# Autodesk Inventor assembly: 2200_Coil Housing
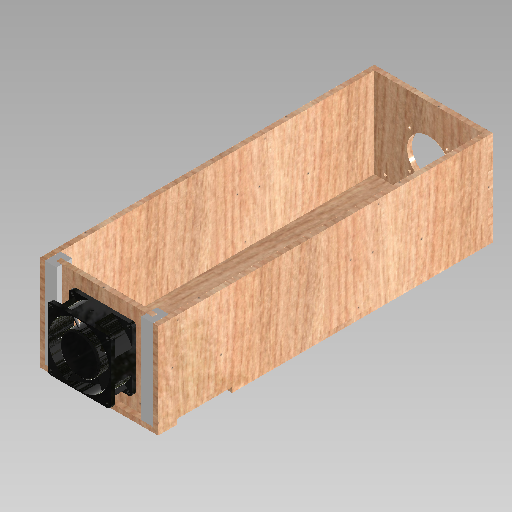
[picture p0: Inventor's stored thumbnail of the model, 512x512]
Saved by Autodesk Inventor 2020 (Build 240168000, 168)
## iProperties
Created: 2019-11-08
Part Number: 2200_Coil Housing
Document SubType Name: Assembly
Designer: RFLab
Author: RFLab
## Documents named in this file (7)
- C:\Users\e22ma\Dropbox\MPI Group Folder\MPS\Inventor_Parts\Parts Numbered - OSMPI\2xxx_Sample Holder and Rx\22xx_Coil Housing\2200_Coil Housing.iam
- C:\Users\e22ma\Dropbox\MPI Group Folder\MPS\Inventor_Parts\Parts Numbered - OSMPI\2xxx_Sample Holder and Rx\22xx_Coil Housing\2204_Housing Front_V1.ipt
- C:\Users\e22ma\Dropbox\MPI Group Folder\MPS\Inventor_Parts\Parts Numbered - OSMPI\2xxx_Sample Holder and Rx\22xx_Coil Housing\2202_Housing Side_V1.ipt
- C:\Users\e22ma\Dropbox\MPI Group Folder\MPS\Inventor_Parts\Parts Numbered - OSMPI\2xxx_Sample Holder and Rx\22xx_Coil Housing\2203_Housing Back.ipt
- C:\Users\e22ma\Dropbox\MPI Group Folder\MPS\Inventor_Parts\Parts Numbered - OSMPI\2xxx_Sample Holder and Rx\22xx_Coil Housing\2208_Back Plate Groove_V1.ipt
- C:\Users\e22ma\Dropbox\MPI Group Folder\MPS\Inventor_Parts\Parts Numbered - OSMPI\2xxx_Sample Holder and Rx\22xx_Coil Housing\2201_Housing Bottom_V1.ipt
- C:\Users\e22ma\Dropbox\MPI Student Access\Helpful Files\Inventor\DC EQUIPMENT COOLING FAN_1939K130.ipt
## Components (8 placed, 6 different names)
1. 2204_Housing Front_V1:1 — Flush:1, Mate:3, Mate:4, Flush:2, Mate:9, Flush:17
2. 2202_Housing Side_V1:1 — Flush:1, Flush:11, Mate:9, Mate:10, Flush:13, Mate:13, Flush:15
3. 2202_Housing Side_V1:2 — Mate:3, Mate:4, Flush:2, Mate:8, Flush:10, Mate:12, Flush:12, Flush:14, Flush:16
4. 2201_Housing Bottom_V1:1 — Mate:8, Flush:10, Flush:11, Mate:10, Mate:11, Flush:17
5. 2203_Housing Back:1 — Mate:11, Mate:14, Flush:16, Mate:15, Mate:16, Mate:17, Mate:18
6. 2208_Back Plate Groove_V1:1 — Mate:12, Flush:12, Flush:14, Mate:14, Mate:15
7. 2208_Back Plate Groove_V1:2 — Flush:13, Mate:13, Flush:15
8. DC EQUIPMENT COOLING FAN_1939K130:1 — Mate:16, Mate:17, Mate:18
## Relationships (23: Mate 13, Flush 10)
- Flush:1: 2204_Housing Front_V1:1 ↔ 2202_Housing Side_V1:1
- Mate:3: 2204_Housing Front_V1:1 ↔ 2202_Housing Side_V1:2
- Mate:4: 2204_Housing Front_V1:1 ↔ 2202_Housing Side_V1:2
- Flush:2: 2204_Housing Front_V1:1 ↔ 2202_Housing Side_V1:2
- Mate:8: 2202_Housing Side_V1:2 ↔ 2201_Housing Bottom_V1:1
- Flush:10: 2202_Housing Side_V1:2 ↔ 2201_Housing Bottom_V1:1
- Flush:11: 2202_Housing Side_V1:1 ↔ 2201_Housing Bottom_V1:1
- Mate:9: 2204_Housing Front_V1:1 ↔ 2202_Housing Side_V1:1
- Mate:10: 2202_Housing Side_V1:1 ↔ 2201_Housing Bottom_V1:1
- Mate:11: 2201_Housing Bottom_V1:1 ↔ 2203_Housing Back:1
- Mate:12: 2202_Housing Side_V1:2 ↔ 2208_Back Plate Groove_V1:1
- Flush:12: 2202_Housing Side_V1:2 ↔ 2208_Back Plate Groove_V1:1
- Flush:13: 2202_Housing Side_V1:1 ↔ 2208_Back Plate Groove_V1:2
- Mate:13: 2202_Housing Side_V1:1 ↔ 2208_Back Plate Groove_V1:2
- Flush:14: 2202_Housing Side_V1:2 ↔ 2208_Back Plate Groove_V1:1
- Flush:15: 2202_Housing Side_V1:1 ↔ 2208_Back Plate Groove_V1:2
- Mate:14: 2203_Housing Back:1 ↔ 2208_Back Plate Groove_V1:1
- Flush:16: 2202_Housing Side_V1:2 ↔ 2203_Housing Back:1
- Mate:15: 2203_Housing Back:1 ↔ 2208_Back Plate Groove_V1:1
- Flush:17: 2204_Housing Front_V1:1 ↔ 2201_Housing Bottom_V1:1
- Mate:16: 2203_Housing Back:1 ↔ DC EQUIPMENT COOLING FAN_1939K130:1
- Mate:17: 2203_Housing Back:1 ↔ DC EQUIPMENT COOLING FAN_1939K130:1
- Mate:18: 2203_Housing Back:1 ↔ DC EQUIPMENT COOLING FAN_1939K130:1
